# Autodesk Inventor assembly: v-166-1a5_r_
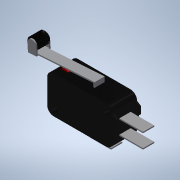
[picture p0: Inventor's stored thumbnail of the model, 180x180]
Saved by Autodesk Inventor 2021 (Build 250183000, 183)
## iProperties
Company: TraceParts S.A.
Created: 2021-06-21
Part Number: v-166-1a5_r_
Checked By: TraceParts S.A.
Catalog Web Link: www.traceparts.com
Document SubType Name: Assembly
Designer: TraceParts
SUPPLIER_NAME: RS Components
SUPPLIER: Omron
DESIGN: Microinterruptor, Palanca de Rodillo SPDT 16 A a 250 V ac
REFERENCE: V-166-1A5(R)
Buy_Now: https://uk.rs-online.com/web/p/products/6822815?cm_mmc=en-ds-_-mcad-_-traceparts-_-6822815'
rs_stock_number: 6822815
TraceParts.PartVersion: 1.0.7
TraceParts.PartStatus: Published
TraceParts.PartNumber: 10-12112013-124526
TraceParts.PartLanguage: es
TraceParts.InstanceId: 10-12112013-1245263JM4Z3NPECSNL38XOL764V6HN
TraceParts.PartTitle: Microinterruptor, Palanca de Rodillo SPDT 16 A a 250 V ac
TRACEPARTS: TRACEPARTS
TraceParts.ClassPath: RS_COMPONENTS:10-12112013-124526
Author: TraceParts
## Documents named in this file (3)
- D:\Nelson\Documentos\Inventor\Proyecto_PAI\v-166-1a5_r_.iam
- D:\Nelson\Documentos\Inventor\Proyecto_PAI\v-166-1a5_r__01.ipt
- D:\Nelson\Documentos\Inventor\Proyecto_PAI\v-166-1a5_r__02.ipt
## Components (2 placed, 2 different names)
1. v-166-1a5_r__01:1 — Mate:1, Flush:1, Flush:2
2. v-166-1a5_r__02:1 — Mate:1, Flush:1, Flush:2
## Relationships (3: Flush 2, Mate 1)
- Mate:1: v-166-1a5_r__01:1 ↔ v-166-1a5_r__02:1
- Flush:1 (16.4 mm): v-166-1a5_r__01:1 ↔ v-166-1a5_r__02:1
- Flush:2 (3.2 mm): v-166-1a5_r__01:1 ↔ v-166-1a5_r__02:1
